# Autodesk Inventor assembly: Сборка2
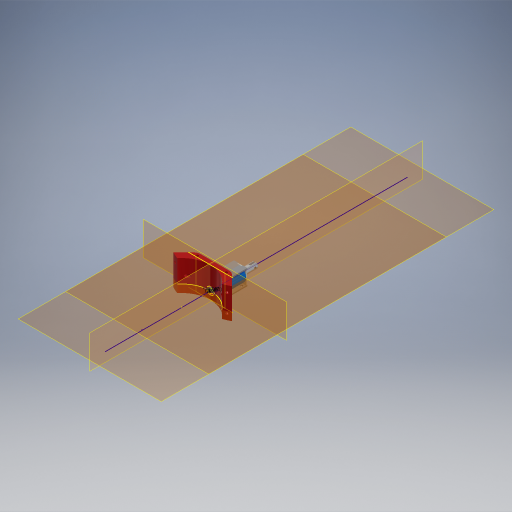
[picture p0: Inventor's stored thumbnail of the model, 512x512]
Saved by Autodesk Inventor 2023 (Build 270158000, 158)
## iProperties
Created: 2025-02-22
Part Number: Сборка2
Document SubType Name: Assembly
Designer: Ivan
Author: Ivan
## Documents named in this file (4)
- C:\!projects\DASH-\3D\Dash-V1\Solenoid\Сборка2.iam
- C:\!projects\DASH-\3D\Dash-V1\catch_v2.ipt
- C:\!projects\DASH-\3D\Dash-V1\Solenoid\Solenoid.iam
- C:\!projects\DASH-\3D\Dash-V1\Solenoid\kick_panel.ipt
## Components (3 placed, 3 different names)
1. catch_v2:1 — Совмещение:1, Совмещение:2, Угол:1, Совмещение:3, Совмещение:4, Угол:2, Совмещение:5, Угол:3, Угол:4
2. Solenoid:1 [sub-assembly] — Совмещение:3, Совмещение:4, Угол:2, Совмещение:6
3. kick_panel:1 — Заподлицо:1, Заподлицо:2, Заподлицо:3
## Relationships (13: Mate 6, Angle 4, Flush 3)
- Совмещение:1 [Mate]: catch_v2:1
- Совмещение:2 [Mate]: catch_v2:1
- Угол:1 [Angle] (0 deg): catch_v2:1
- Совмещение:3 [Mate] (2.663 mm): catch_v2:1 ↔ Solenoid:1
- Совмещение:4 [Mate]: catch_v2:1 ↔ Solenoid:1
- Угол:2 [Angle] (0 deg): catch_v2:1 ↔ Solenoid:1
- Совмещение:5 [Mate]: catch_v2:1
- Угол:3 [Angle] (0 deg): catch_v2:1
- Заподлицо:1 [Flush]: kick_panel:1
- Заподлицо:2 [Flush]: kick_panel:1
- Совмещение:6 [Mate]: Solenoid:1
- Угол:4 [Angle] (0 deg): catch_v2:1
- Заподлицо:3 [Flush]: kick_panel:1
